# Autodesk Inventor assembly: FemPodstawa
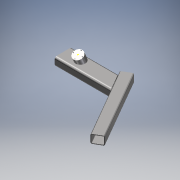
[picture p0: Inventor's stored thumbnail of the model, 180x180]
Saved by Autodesk Inventor 2017 (Build 210142000, 142)
## iProperties
Created: 2016-12-08
Part Number: FemPodstawa
Document SubType Name: Assembly
Designer: Marcin
Mass: 27254.7 g
Surface Area: 9371.53 cm^2
Volume: 3503.65 cm^3
Density: 7.77893 g/cm^3
Author: Marcin
## Documents named in this file (11)
- M:\PracaInżynierska\FEM\FemPodstawa.iam
- M:\PracaInżynierska\PodstawaFem.ipt
- M:\PracaInżynierska\WynikiZadaniaOdwrotnego\PN EN 10219-2 - 100 x 80 x 6  - 655.ipt
- M:\PracaInżynierska\WynikiZadaniaOdwrotnego\PN EN 10219-2 - 160 x 80 x 8  - 545.ipt
- M:\PracaInżynierska\WynikiZadaniaOdwrotnego\PN EN 10060 - 75 - 50.ipt
- M:\PracaInżynierska\FEM\FemPodstawa\AIP\FEA\bznybyl28.fins
- M:\PracaInżynierska\FEM\FemPodstawa\AIP\FEA\bznybyl28.fsat
- M:\PracaInżynierska\FEM\FemPodstawa\AIP\FEA\bznybyl28.ftes
- M:\PracaInżynierska\FEM\FemPodstawa\AIP\FEA\bznybyl28.fwiz
- M:\PracaInżynierska\FEM\FemPodstawa\AIP\FEA\bznybyl40.fmsh
- M:\PracaInżynierska\FEM\FemPodstawa\AIP\FEA\bznybyl41.fres
## Components (4 placed, 4 different names)
1. PodstawaFem:1 — Flush:13
2. PN EN 10219-2 - 100 x 80 x 6  - 655:1 — Mate:3, Flush:5
3. PN EN 10219-2 - 160 x 80 x 8  - 545:1 — Mate:3, Flush:5, Mate:4
4. PodSilownik — Mate:4, Flush:13
## Relationships (6: Flush 4, Mate 2)
- Mate:3: PN EN 10219-2 - 100 x 80 x 6  - 655:1 ↔ PN EN 10219-2 - 160 x 80 x 8  - 545:1
- Flush:5: PN EN 10219-2 - 100 x 80 x 6  - 655:1 ↔ PN EN 10219-2 - 160 x 80 x 8  - 545:1
- Mate:4: PN EN 10219-2 - 160 x 80 x 8  - 545:1 ↔ PodSilownik
- [Flush]: PodstawaFem:1 ↔ PodSilownik
- [Flush]: PodstawaFem:1 ↔ PodSilownik
- Flush:13: PodstawaFem:1 ↔ PodSilownik
## Named parameters: sa_0 = 17421.6, sa_1 = 362523, sa_2 = 168147
note: some values were not read from the file. Shown as the stored number, unit unknown: "sa_0", "sa_1", "sa_2".
